# Autodesk Inventor assembly: BridWaterAssembly
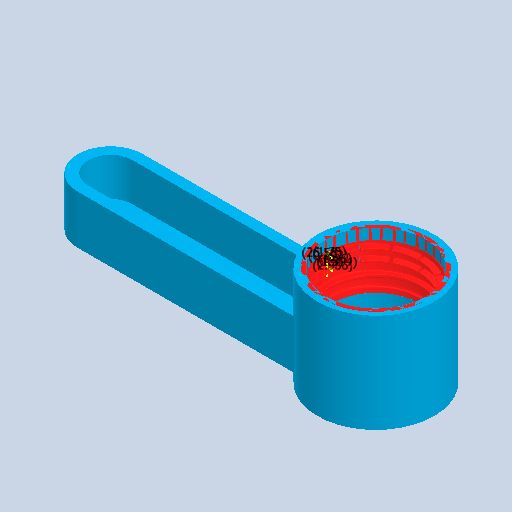
[picture p0: Inventor's stored thumbnail of the model, 512x512]
Saved by Autodesk Inventor 2022.1 (Build 261234020, 234B)
## iProperties
Created: 2021-10-29
Part Number: BridWaterAssembly
Document SubType Name: Assembly
Designer: robst
Author: robst
## Documents named in this file (3)
- C:\git\CAD-Development\robSteele\HouseProjects\Bird\BridWaterAssembly.iam
- C:\git\CAD-Development\robSteele\HouseProjects\Bird\birdWaterForCageAttachement.ipt
- C:\git\CAD-Development\robSteele\HouseProjects\Bird\Red_bottle_cap.ipt
## Components (2 placed, 2 different names)
1. birdWaterForCageAttachement:1 — Insert:1
2. Red_bottle_cap:1 — Insert:1
## Relationships (1: Insert 1)
- Insert:1: birdWaterForCageAttachement:1 ↔ Red_bottle_cap:1
